# Autodesk Inventor assembly: cylinder assembly
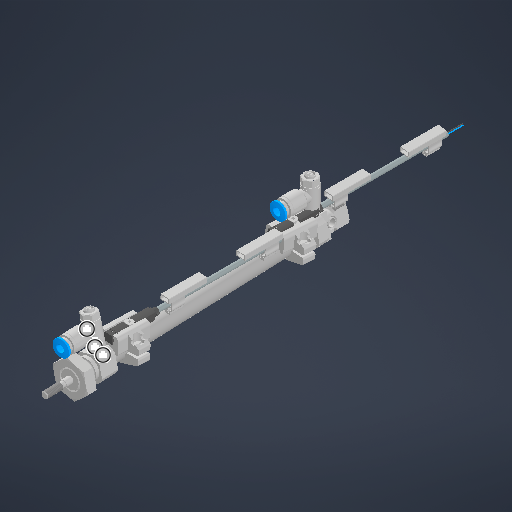
[picture p0: Inventor's stored thumbnail of the model, 512x512]
Saved by Autodesk Inventor 2027 (Build 310192000, 192)
## iProperties
Created: 2026-04-16
Part Number: cylinder assembly
Document SubType Name: Assembly
Designer: ratik
Author: ratik
## Documents named in this file (5)
- C:\Users\ratik\OneDrive\Personal Folder\00_Startup\01_Mectosys_Prototype\01_Prototype\01_Mechanical\3D file\04_Distribution module\Cylinder assembly\cylinder assembly.iam
- C:\Users\ratik\OneDrive\Personal Folder\00_Startup\01_Mectosys_Prototype\01_Prototype\01_Mechanical\3D file\04_Distribution module\35_PARTserver0202604161719057653412610e898ce\AIS2024\19182 DSNU-8-100-P-A---(0).iam
- C:\Users\ratik\OneDrive\Personal Folder\00_Startup\01_Mectosys_Prototype\01_Prototype\01_Mechanical\3D file\04_Distribution module\36_PARTserver0202604161723152183443510e898ce\AIS2024\574335 SMT-8M-A-PS-24V-E-2,5-OE.iam
- C:\Users\ratik\OneDrive\Personal Folder\00_Startup\01_Mectosys_Prototype\01_Prototype\01_Mechanical\3D file\04_Distribution module\37_PARTserver0202604161726300103468710e898ce\175091 SMBR-8-8.ipt
- C:\Users\ratik\OneDrive\Personal Folder\00_Startup\01_Mectosys_Prototype\01_Prototype\01_Mechanical\3D file\04_Distribution module\38_PARTserver0202604161737460883546210e898ce\193138 GRLA-M5-QS-4-D.ipt
## Components (7 placed, 4 different names)
1. 19182 DSNU-8-100-P-A---(0):1 [sub-assembly] — Mate:1, Mate:2, Mate:3, Mate:4
2. 574335 SMT-8M-A-PS-24V-E-2,5-OE:1 [sub-assembly] — Mate:5
3. 175091 SMBR-8-8:1 — Mate:1, Mate:5
4. 193138 GRLA-M5-QS-4-D:1 — Mate:3
5. 175091 SMBR-8-8:2 — Mate:2, Mate:6
6. 193138 GRLA-M5-QS-4-D:2 — Mate:4
7. 574335 SMT-8M-A-PS-24V-E-2,5-OE:2 [sub-assembly] — Mate:6
## Relationships (6: Mate 6)
- Mate:1: 19182 DSNU-8-100-P-A---(0):1 ↔ 175091 SMBR-8-8:1
- Mate:2: 19182 DSNU-8-100-P-A---(0):1 ↔ 175091 SMBR-8-8:2
- Mate:3: 19182 DSNU-8-100-P-A---(0):1 ↔ 193138 GRLA-M5-QS-4-D:1
- Mate:4: 19182 DSNU-8-100-P-A---(0):1 ↔ 193138 GRLA-M5-QS-4-D:2
- Mate:5: 574335 SMT-8M-A-PS-24V-E-2,5-OE:1 ↔ 175091 SMBR-8-8:1
- Mate:6: 175091 SMBR-8-8:2 ↔ 574335 SMT-8M-A-PS-24V-E-2,5-OE:2
